# Autodesk Inventor assembly: testing
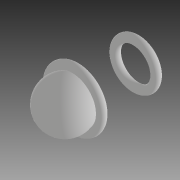
[picture p0: Inventor's stored thumbnail of the model, 180x180]
Saved by Autodesk Inventor 2020 (Build 240168000, 168)
## iProperties
Created: 2020-11-28
Part Number: testing
Document SubType Name: Assembly
Designer: DDeGo
Author: DDeGo
## Documents named in this file (5)
- C:\Users\DDeGo\Documents\Drew\Projects\AirWankelEngine\cad\testing.iam
- C:\Users\DDeGo\Documents\Drew\Projects\AirWankelEngine\cad\6mm bb.ipt
- C:\Users\DDeGo\Documents\Drew\Projects\AirWankelEngine\cad\oring_4x6.ipt
- C:\Users\DDeGo\Documents\Drew\Projects\AirWankelEngine\cad\oring_5x7.ipt
- C:\Users\DDeGo\Documents\Drew\Projects\AirWankelEngine\cad\oring_5p5x7p5.ipt
## Components (4 placed, 4 different names)
1. 6mm bb:1 — Mate:1, Mate:2, Mate:3
2. oring_4x6:1 — Mate:1, Angle:6
3. oring_5x7:1 — Mate:2, Angle:5
4. oring_5p5x7p5:1 — Angle:7, Mate:3
## Relationships (6: Mate 3, Angle 3)
- Mate:1: 6mm bb:1 ↔ oring_4x6:1
- Mate:2: 6mm bb:1 ↔ oring_5x7:1
- Angle:6 (0 deg): oring_4x6:1
- Angle:5 (0 deg): oring_5x7:1
- Angle:7 (0 deg): oring_5p5x7p5:1
- Mate:3: 6mm bb:1 ↔ oring_5p5x7p5:1
